# Autodesk Inventor assembly: POM_T5_05
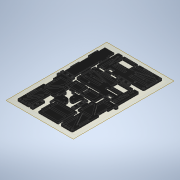
[picture p0: Inventor's stored thumbnail of the model, 180x180]
Saved by Autodesk Inventor 2020 (Build 240168000, 168)
## iProperties
Created: 2021-08-27
Part Number: POM_T5_05
Document SubType Name: Assembly
Designer: Masato
Author: Masato
## Documents named in this file (12)
- C:\Users\naoki\Documents\Inventor\CitBrains\git_clone\OpenPlatform4_0\再切削_POM_T5\OpenPlatform_ver3_0\cam\POM_T5_05.iam
- C:\Users\naoki\Documents\Inventor\CitBrains\git_clone\OpenPlatform4_0\コックピットCAM\OpenPlatform_ver3_0\cam\Disposable_Board.ipt
- C:\Users\naoki\Documents\Inventor\CitBrains\git_clone\OpenPlatform4_0\再切削_POM_T5\OpenPlatform_ver3_0\UpperBody\Cockpit\Cockpit_lower_back_door.ipt
- C:\Users\naoki\Documents\Inventor\CitBrains\git_clone\OpenPlatform4_0\再切削_POM_T5\OpenPlatform_ver3_0\UpperBody\Cockpit\Cockpit_lower_bottom_frame.ipt
- C:\Users\naoki\Documents\Inventor\CitBrains\git_clone\OpenPlatform4_0\再切削_POM_T5\OpenPlatform_ver3_0\UpperBody\Cockpit\Cockpit_lower_front_frame.ipt
- C:\Users\naoki\Documents\Inventor\CitBrains\git_clone\OpenPlatform4_0\再切削_POM_T5\OpenPlatform_ver3_0\UpperBody\Cockpit\Cockpit_lower_side_frame.ipt
- C:\Users\naoki\Documents\Inventor\CitBrains\git_clone\OpenPlatform4_0\再切削_POM_T5\OpenPlatform_ver3_0\UpperBody\Cockpit\Cockpit_lower_side_frame_MIR.ipt
- C:\Users\naoki\Documents\Inventor\CitBrains\git_clone\OpenPlatform4_0\再切削_POM_T5\OpenPlatform_ver3_0\UpperBody\Cockpit\Cockpit_upper_front_frame.ipt
- C:\Users\naoki\Documents\Inventor\CitBrains\git_clone\OpenPlatform4_0\再切削_POM_T5\OpenPlatform_ver3_0\UpperBody\Trunk\Trunk_abdomen_spacer.ipt
- C:\Users\naoki\Documents\Inventor\CitBrains\git_clone\OpenPlatform4_0\再切削_POM_T5\OpenPlatform_ver3_0\UpperBody\Head\Camera_side_frame.ipt
- C:\Users\naoki\Documents\Inventor\CitBrains\git_clone\OpenPlatform4_0\再切削_POM_T5\OpenPlatform_ver3_0\UpperBody\Cockpit\Cockpit_upper_side_frame.ipt
- C:\Users\naoki\Documents\Inventor\CitBrains\git_clone\OpenPlatform4_0\再切削_POM_T5\OpenPlatform_ver3_0\UpperBody\Cockpit\Cockpit_upper_side_frame_MIR.ipt
## Components (15 placed, 11 different names)
1. Disposable_Board:1 — メイト:2, メイト:1, フラッシュ:1, フラッシュ:2, フラッシュ:3, フラッシュ:8, フラッシュ:9, フラッシュ:10, メイト:26, メイト:27, フラッシュ:15
2. Cockpit_lower_back_door:1 — メイト:5, メイト:10, メイト:30, メイト:35, メイト:36
3. Cockpit_lower_bottom_frame:1 — メイト:6, メイト:38, メイト:39, メイト:40, フラッシュ:15
4. Cockpit_lower_front_frame:1 — メイト:9, メイト:28, メイト:32, メイト:33
5. Cockpit_lower_side_frame:1 — メイト:4, フラッシュ:3, フラッシュ:8, メイト:25, メイト:32, フラッシュ:14, メイト:37, メイト:41
6. Cockpit_lower_side_frame_MIR:1 — メイト:8, フラッシュ:9, フラッシュ:13, メイト:24, メイト:29, メイト:30
7. Cockpit_upper_front_frame:1 — メイト:7, フラッシュ:10, フラッシュ:13, メイト:23, メイト:29, 正接:3
8. Trunk_abdomen_spacer:1 — メイト:14, フラッシュ:14, メイト:37, メイト:38
9. Trunk_abdomen_spacer:2 — メイト:15, メイト:42, メイト:43
10. Trunk_abdomen_spacer:3 — メイト:13, メイト:23, メイト:24
11. Trunk_abdomen_spacer:4 — メイト:11, メイト:41
12. Camera_side_frame:1 — メイト:25, メイト:26, 正接:2, 正接:3
13. Camera_side_frame:2 — メイト:27, 正接:2, メイト:28
14. Cockpit_upper_side_frame:1 — メイト:22, メイト:33, メイト:34, メイト:35, メイト:36, メイト:39, メイト:42
15. Cockpit_upper_side_frame_MIR:1 — メイト:21, メイト:34, メイト:40, メイト:43
## Relationships (46: Mate 35, Flush 9, Tangent 2)
- メイト:2 [Mate]: Disposable_Board:1
- メイト:1 [Mate]: Disposable_Board:1
- フラッシュ:1 [Flush]: Disposable_Board:1
- フラッシュ:2 [Flush]: Disposable_Board:1
- メイト:4 [Mate]: Cockpit_lower_side_frame:1
- メイト:5 [Mate]: Cockpit_lower_back_door:1
- メイト:6 [Mate]: Cockpit_lower_bottom_frame:1
- メイト:7 [Mate]: Cockpit_upper_front_frame:1
- メイト:8 [Mate]: Cockpit_lower_side_frame_MIR:1
- メイト:9 [Mate]: Cockpit_lower_front_frame:1
- メイト:10 [Mate]: Cockpit_lower_back_door:1
- メイト:11 [Mate]: Trunk_abdomen_spacer:4
- メイト:13 [Mate]: Trunk_abdomen_spacer:3
- メイト:14 [Mate]: Trunk_abdomen_spacer:1
- メイト:15 [Mate]: Trunk_abdomen_spacer:2
- メイト:21 [Mate]: Cockpit_upper_side_frame_MIR:1
- メイト:22 [Mate]: Cockpit_upper_side_frame:1
- フラッシュ:3 [Flush] (2 mm): Disposable_Board:1 ↔ Cockpit_lower_side_frame:1
- フラッシュ:8 [Flush] (2 mm): Disposable_Board:1 ↔ Cockpit_lower_side_frame:1
- フラッシュ:9 [Flush] (2.5 mm): Disposable_Board:1 ↔ Cockpit_lower_side_frame_MIR:1
- フラッシュ:10 [Flush] (2 mm): Disposable_Board:1 ↔ Cockpit_upper_front_frame:1
- フラッシュ:13 [Flush]: Cockpit_lower_side_frame_MIR:1 ↔ Cockpit_upper_front_frame:1
- メイト:23 [Mate] (2.5 mm): Cockpit_upper_front_frame:1 ↔ Trunk_abdomen_spacer:3
- メイト:24 [Mate] (2.5 mm): Cockpit_lower_side_frame_MIR:1 ↔ Trunk_abdomen_spacer:3
- メイト:25 [Mate] (2.5 mm): Cockpit_lower_side_frame:1 ↔ Camera_side_frame:1
- メイト:26 [Mate]: Disposable_Board:1 ↔ Camera_side_frame:1
- メイト:27 [Mate]: Disposable_Board:1 ↔ Camera_side_frame:2
- 正接:2 [Tangent] (2.5 mm): Camera_side_frame:1 ↔ Camera_side_frame:2
- メイト:28 [Mate] (2.5 mm): Cockpit_lower_front_frame:1 ↔ Camera_side_frame:2
- メイト:29 [Mate] (2.5 mm): Cockpit_lower_side_frame_MIR:1 ↔ Cockpit_upper_front_frame:1
- メイト:30 [Mate] (2.5 mm): Cockpit_lower_back_door:1 ↔ Cockpit_lower_side_frame_MIR:1
- メイト:32 [Mate] (2.5 mm): Cockpit_lower_front_frame:1 ↔ Cockpit_lower_side_frame:1
- メイト:33 [Mate] (2.5 mm): Cockpit_lower_front_frame:1 ↔ Cockpit_upper_side_frame:1
- メイト:34 [Mate] (4.5 mm): Cockpit_upper_side_frame:1 ↔ Cockpit_upper_side_frame_MIR:1
- メイト:35 [Mate] (2.5 mm): Cockpit_lower_back_door:1 ↔ Cockpit_upper_side_frame:1
- メイト:36 [Mate] (2.5 mm): Cockpit_lower_back_door:1 ↔ Cockpit_upper_side_frame:1
- フラッシュ:14 [Flush]: Cockpit_lower_side_frame:1 ↔ Trunk_abdomen_spacer:1
- メイト:37 [Mate] (2.5 mm): Cockpit_lower_side_frame:1 ↔ Trunk_abdomen_spacer:1
- メイト:38 [Mate] (2.5 mm): Cockpit_lower_bottom_frame:1 ↔ Trunk_abdomen_spacer:1
- メイト:39 [Mate] (2.5 mm): Cockpit_lower_bottom_frame:1 ↔ Cockpit_upper_side_frame:1
- メイト:40 [Mate] (2.5 mm): Cockpit_lower_bottom_frame:1 ↔ Cockpit_upper_side_frame_MIR:1
- フラッシュ:15 [Flush] (2 mm): Disposable_Board:1 ↔ Cockpit_lower_bottom_frame:1
- メイト:41 [Mate] (2.5 mm): Cockpit_lower_side_frame:1 ↔ Trunk_abdomen_spacer:4
- 正接:3 [Tangent] (-2.5 mm): Cockpit_upper_front_frame:1 ↔ Camera_side_frame:1
- メイト:42 [Mate] (2.25 mm): Trunk_abdomen_spacer:2 ↔ Cockpit_upper_side_frame:1
- メイト:43 [Mate] (3 mm): Trunk_abdomen_spacer:2 ↔ Cockpit_upper_side_frame_MIR:1
